# Autodesk Inventor assembly: center_holder
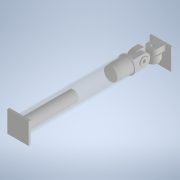
[picture p0: Inventor's stored thumbnail of the model, 180x180]
Saved by Autodesk Inventor 2020 (Build 240168000, 168)
## iProperties
Created: 2019-04-30
Part Number: center_holder
Document SubType Name: Assembly
Designer: erwin
Author: erwin
## Documents named in this file (7)
- D:\GitHub\DrowningWarnings\wave_simulator\center_holder.iam
- D:\GitHub\DrowningWarnings\wave_simulator\center_holder_top.ipt
- D:\GitHub\DrowningWarnings\wave_simulator\tube.ipt
- D:\GitHub\DrowningWarnings\wave_simulator\center_holder_bottom.ipt
- D:\GitHub\DrowningWarnings\wave_simulator\center_holder_top_center.ipt
- D:\GitHub\DrowningWarnings\wave_simulator\center_holder_boat.ipt
- D:\GitHub\DrowningWarnings\wave_simulator\center_holder_retainer.ipt
## Components (6 placed, 6 different names)
1. center_holder_top:1 — Flush:1, Flush:3
2. tube:1 — Flush:1, Flush:2
3. center_holder_bottom:1 — Flush:2
4. center_holder_top_center:1 — Flush:3, Flush:4
5. center_holder_boat:1 — Flush:4, Flush:5
6. center_holder_retainer:1 — Flush:5
## Relationships (5: Flush 5)
- Flush:1: center_holder_top:1 ↔ tube:1
- Flush:2: tube:1 ↔ center_holder_bottom:1
- Flush:3 (0.5 mm): center_holder_top:1 ↔ center_holder_top_center:1
- Flush:4: center_holder_top_center:1 ↔ center_holder_boat:1
- Flush:5: center_holder_boat:1 ↔ center_holder_retainer:1
